# Autodesk Inventor assembly: Existing_Kitchen_And_Dining_Room
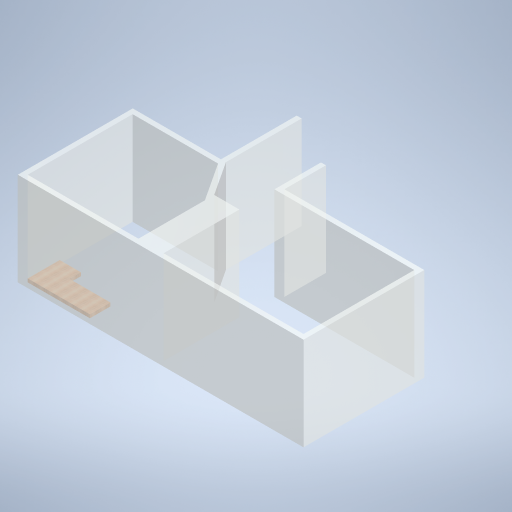
[picture p0: Inventor's stored thumbnail of the model, 512x512]
Saved by Autodesk Inventor 2024 (Build 280153000, 153)
## iProperties
Created: 2023-05-06
Part Number: Existing_Kitchen_And_Dining_Room
Document SubType Name: Assembly
Designer: Tom
Author: Tom
## Documents named in this file (3)
- C:\Users\Tom\Documents\Tom_Levers_Public_Git_Repository\Inventor\House\Existing_Kitchen_And_Dining_Room.iam
- C:\Users\Tom\Documents\Tom_Levers_Public_Git_Repository\Inventor\House\Existing_Kitchen_And_Dining_Room.ipt
- C:\Users\Tom\Documents\Tom_Levers_Public_Git_Repository\Inventor\House\Stand--Sink_and_Corner_Cabinets.ipt
## Components (2 placed, 2 different names)
1. Existing_Kitchen_And_Dining_Room:1 — Mate:1, Mate:2, Flush:1
2. Stand--Sink_and_Corner_Cabinets:1 — Mate:1, Mate:2, Flush:1
## Relationships (3: Mate 2, Flush 1)
- Mate:1: Existing_Kitchen_And_Dining_Room:1 ↔ Stand--Sink_and_Corner_Cabinets:1
- Mate:2: Existing_Kitchen_And_Dining_Room:1 ↔ Stand--Sink_and_Corner_Cabinets:1
- Flush:1: Existing_Kitchen_And_Dining_Room:1 ↔ Stand--Sink_and_Corner_Cabinets:1
